# Autodesk Inventor assembly: Combined
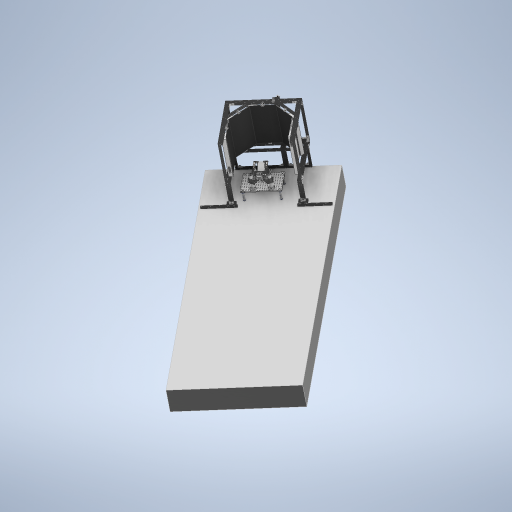
[picture p0: Inventor's stored thumbnail of the model, 512x512]
Saved by Autodesk Inventor 2024 (Build 280153000, 153)
## iProperties
Created: 2021-10-11
Part Number: Combined
Document SubType Name: Assembly
Designer: gnzak
Author: gnzak
## Documents named in this file (8)
- C:\Users\rosam\OneDrive\Documents\github_latest\Hardware\Tablet-Rig\Assemblies\Combined_imaging.iam
- C:\Users\rosam\OneDrive\Documents\github_latest\Hardware\Tablet-Rig\Parts\Table.ipt
- C:\Users\rosam\OneDrive\Documents\github_latest\Hardware\Tablet-Rig\Parts\Objective Location Marker.ipt
- C:\Users\rosam\OneDrive\Documents\github_latest\Hardware\Tablet-Rig\Assemblies\Frame_imaging.iam
- C:\Users\rosam\OneDrive\Documents\github_latest\Hardware\Tablet-Rig\Parts\ThorLabs RS020\RS020-Step.ipt
- C:\Users\rosam\OneDrive\Documents\github_latest\Hardware\Tablet-Rig\Parts\ThorLabs RS4\RS4-Step.ipt
- C:\Users\rosam\OneDrive\Documents\github_latest\Hardware\Tablet-Rig\Parts\ThorLabs RS1\RS1-Step.ipt
- C:\Users\rosam\OneDrive\Documents\github_latest\Hardware\Tablet-Rig\Assemblies\Wheel_w_board_rotatable.iam
## Components (16 placed, 7 different names)
1. Table:1 — Mate:26, Flush:14, Mate:27, Flush:50, Mate:140, Mate:141, Mate:142, Mate:143, Angle:1, Angle:2
2. Objective Location Marker:1 — Mate:26, Flush:14, Mate:27, Mate:98, Flush:49, Mate:99, Mate:149, Flush:51
3. Frame_imaging:1 [sub-assembly] — Mate:98, Flush:49, Mate:99
4. RS020-Step:5 — Mate:140
5. RS4-Step:5 — Mate:145
6. RS1-Step:5
7. RS020-Step:6 — Mate:141
8. RS4-Step:6 — Mate:146
9. RS1-Step:6 — Mate:148
10. RS020-Step:7 — Mate:142
11. RS4-Step:7 — Mate:147
12. RS1-Step:7
13. RS020-Step:8 — Mate:143
14. RS4-Step:8 — Mate:144
15. RS1-Step:8
16. Wheel_w_board_rotatable:1 [sub-assembly] — Angle:1, Angle:2, Mate:144, Mate:145, Mate:146, Mate:147, Mate:148, Mate:149, Flush:51
## Relationships (36: Mate 30, Flush 4, Angle 2)
- Mate:26: Table:1 ↔ Objective Location Marker:1
- Flush:14 (355.6 mm): Table:1 ↔ Objective Location Marker:1
- Mate:27 (-755.65 mm): Table:1 ↔ Objective Location Marker:1
- Mate:98 (381 mm): Objective Location Marker:1 ↔ Frame_imaging:1
- Flush:49: Objective Location Marker:1 ↔ Frame_imaging:1
- Mate:99 (-127 mm): Objective Location Marker:1 ↔ Frame_imaging:1
- Flush:50 (-685.8 mm): Table:1
- [Mate]: RS4-Step:5 ↔ RS1-Step:5
- [Mate]: RS020-Step:5 ↔ RS4-Step:5
- [Mate]: RS020-Step:5 ↔ RS4-Step:5
- [Mate]: RS4-Step:5 ↔ RS1-Step:5
- [Mate]: RS4-Step:6 ↔ RS1-Step:6
- [Mate]: RS020-Step:6 ↔ RS4-Step:6
- [Mate]: RS020-Step:6 ↔ RS4-Step:6
- [Mate]: RS4-Step:6 ↔ RS1-Step:6
- [Mate]: RS4-Step:7 ↔ RS1-Step:7
- [Mate]: RS020-Step:7 ↔ RS4-Step:7
- [Mate]: RS020-Step:7 ↔ RS4-Step:7
- [Mate]: RS4-Step:7 ↔ RS1-Step:7
- [Mate]: RS4-Step:8 ↔ RS1-Step:8
- [Mate]: RS020-Step:8 ↔ RS4-Step:8
- [Mate]: RS020-Step:8 ↔ RS4-Step:8
- [Mate]: RS4-Step:8 ↔ RS1-Step:8
- Mate:140: Table:1 ↔ RS020-Step:5
- Mate:141: Table:1 ↔ RS020-Step:6
- Mate:142: Table:1 ↔ RS020-Step:7
- Mate:143: Table:1 ↔ RS020-Step:8
- Angle:1 (0 deg): Table:1 ↔ Wheel_w_board_rotatable:1
- Angle:2 (0 deg): Table:1 ↔ Wheel_w_board_rotatable:1
- Mate:144: RS4-Step:8 ↔ Wheel_w_board_rotatable:1
- Mate:145: RS4-Step:5 ↔ Wheel_w_board_rotatable:1
- Mate:146: RS4-Step:6 ↔ Wheel_w_board_rotatable:1
- Mate:147: RS4-Step:7 ↔ Wheel_w_board_rotatable:1
- Mate:148: RS1-Step:6 ↔ Wheel_w_board_rotatable:1
- Mate:149: Objective Location Marker:1 ↔ Wheel_w_board_rotatable:1
- Flush:51 (91.44 mm): Objective Location Marker:1 ↔ Wheel_w_board_rotatable:1
## Named parameters: d277_d265_d254 = 0 mm, d278_d266_d255 = 0 mm, d279_d267_d252 = 0 mm, d280_d268_d253 = 0 mm, d281_d277_d265_d254 = 0 mm, d282_d278_d266_d255 = 0 mm, d283_d279_d267_d252 = 0 mm, d284_d280_d268_d253 = 0 mm, d285_d277_d265_d254 = 0 mm, d286_d278_d266_d255 = 0 mm, d287_d279_d267_d252 = 0 mm, d288_d280_d268_d253 = 0 mm, d289_d277_d265_d254 = 0 mm, d290_d278_d266_d255 = 0 mm, d291_d279_d267_d252 = 0 mm, d292_d280_d268_d253 = 0 mm
